# Autodesk Inventor assembly: tensor
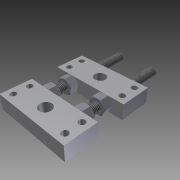
[picture p0: Inventor's stored thumbnail of the model, 180x180]
Saved by Autodesk Inventor 2011 (Build 150239000, 239)
## iProperties
Created: 2010-04-23
Part Number: tensor
Document SubType Name: Assembly
Designer: lucio
Author: lucio
## Documents named in this file (4)
- C:\Users\lucio\Documents\Inventor\caterpillar\tensor.iam
- C:\Users\lucio\Documents\Inventor\caterpillar\montura tensor.ipt
- C:\Users\lucio\Documents\Inventor\caterpillar\barra tensor.ipt
- C:\Users\lucio\Documents\Inventor\Content Center Files\R2011\en-US\ANSI B 18.2.4.1 M(1)\ANSI B 18.2.4.1 M - M6 x 1Style 2.ipt
## Components (8 placed, 3 different names)
1. montura tensor:1 — Mate:1, Mate:2, Flush:1, Flush:2, Mate:9, Mate:10
2. montura tensor:2 — Mate:3, Mate:4, Mate:11, Mate:12
3. barra tensor:1 — Mate:2, Flush:1, Mate:3, Mate:5, Mate:6
4. barra tensor:2 — Mate:1, Flush:2, Mate:4, Mate:7, Mate:8
5. Hex Nut Metric M6 x 1:1 — Mate:8, Mate:12
6. Hex Nut Metric M6 x 1:2 — Mate:7, Mate:10
7. Hex Nut Metric M6 x 1:3 — Mate:5, Mate:9
8. Hex Nut Metric M6 x 1:4 — Mate:6, Mate:11
## Relationships (14: Mate 12, Flush 2)
- Mate:1: montura tensor:1 ↔ barra tensor:2
- Mate:2: montura tensor:1 ↔ barra tensor:1
- Flush:1: montura tensor:1 ↔ barra tensor:1
- Flush:2: montura tensor:1 ↔ barra tensor:2
- Mate:3: montura tensor:2 ↔ barra tensor:1
- Mate:4: montura tensor:2 ↔ barra tensor:2
- Mate:5: barra tensor:1 ↔ Hex Nut Metric M6 x 1:3
- Mate:6: barra tensor:1 ↔ Hex Nut Metric M6 x 1:4
- Mate:7: barra tensor:2 ↔ Hex Nut Metric M6 x 1:2
- Mate:8: barra tensor:2 ↔ Hex Nut Metric M6 x 1:1
- Mate:9: montura tensor:1 ↔ Hex Nut Metric M6 x 1:3
- Mate:10: montura tensor:1 ↔ Hex Nut Metric M6 x 1:2
- Mate:11: montura tensor:2 ↔ Hex Nut Metric M6 x 1:4
- Mate:12: montura tensor:2 ↔ Hex Nut Metric M6 x 1:1
